# Autodesk Inventor assembly: 17-0028-0036
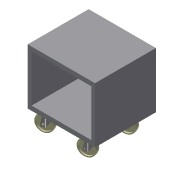
[picture p0: Inventor's stored thumbnail of the model, 180x180]
Saved by Autodesk Inventor 2016 SP2 (Build 200236200, 236)
## iProperties
Category: IOP
Company: Universiteit van Amsterdam
Created: 2017-11-20
Part Number: 17-0028-0036
Document SubType Name: Assembly
Designer: Daan Giesen
Project: Digital PID Loop
Cost Center: 17-0028
User Status: Work in Progress
Authority: Reichsöllner, Lukas
Description: 19" rack 8u
Author: Daan Giesen
Title: Digital PID Loop
Revision Number: A
## Documents named in this file (3)
- D:\VaultLocalWorkingFolder\UvA_MT\Projects\2017\17-0028 Digital PID Loop\20_3D-Models\17-0028-0036.iam
- D:\VaultLocalWorkingFolder\UvA_MT\Projects\2017\17-0028 Digital PID Loop\20_3D-Models\17-0028-0033.ipt
- D:\VaultLocalWorkingFolder\UvA_MT\UVA_library\Wielen\124remwiel.iam
## Components (5 placed, 2 different names)
1. 17-0028-0033:1 — Mate:1, Flush:1, Flush:2
2. 124remwiel:1 [sub-assembly] — Mate:1, Flush:1, Flush:2
3. 124remwiel:2 [sub-assembly]
4. 124remwiel:3 [sub-assembly]
5. 124remwiel:4 [sub-assembly]
## Component patterns: (4 elements, first: 124remwiel:1)
## Relationships (3: Flush 2, Mate 1)
- Mate:1: 17-0028-0033:1 ↔ 124remwiel:1
- Flush:1 (40 mm): 17-0028-0033:1 ↔ 124remwiel:1
- Flush:2 (40 mm): 17-0028-0033:1 ↔ 124remwiel:1
